# Autodesk Inventor assembly: POM_T5_01
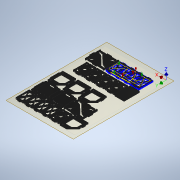
[picture p0: Inventor's stored thumbnail of the model, 180x180]
Saved by Autodesk Inventor 2020 (Build 240168000, 168)
## iProperties
Created: 2021-08-27
Part Number: POM_T5_01
Document SubType Name: Assembly
Designer: Masato
Author: Masato
## Documents named in this file (8)
- C:\Users\L20C1118 森　圭汰\Documents\220317_open\SUSTAINA-OP\Cam\POM_T5_01.iam
- C:\Users\L20C1118 森　圭汰\Documents\220317_open\SUSTAINA-OP\Cam\DisposableBoard.ipt
- C:\Users\L20C1118 森　圭汰\Documents\220317_open\SUSTAINA-OP\UpperBody\Head\Camera_root_frame.ipt
- C:\Users\L20C1118 森　圭汰\Documents\220317_open\SUSTAINA-OP\UpperBody\Head\Head_diagonal.ipt
- C:\Users\L20C1118 森　圭汰\Documents\220317_open\SUSTAINA-OP\UpperBody\Head\Head_horn_frame.ipt
- C:\Users\L20C1118 森　圭汰\Documents\220317_open\SUSTAINA-OP\UpperBody\Arm\ForeArm_diagonal.ipt
- C:\Users\L20C1118 森　圭汰\Documents\220317_open\SUSTAINA-OP\UpperBody\Head\Camera_side_frame.ipt
- C:\Users\L20C1118 森　圭汰\Documents\220317_open\SUSTAINA-OP\SandBlastingJig\Trunk_servo_bottom_frame_SandBlastingJig.ipt
## Components (29 placed, 7 different names)
1. DisposableBoard:1 — メイト:2, メイト:1, フラッシュ:1, フラッシュ:2, フラッシュ:3, フラッシュ:4, メイト:4, メイト:5, メイト:13, メイト:22, メイト:25, メイト:27, メイト:29, フラッシュ:12, フラッシュ:13, メイト:33, メイト:35, メイト:38, メイト:39, メイト:53, メイト:56, メイト:63, メイト:64, メイト:65, メイト:66, メイト:67
2. Camera_root_frame:1 — メイト:27, フラッシュ:11, メイト:41, メイト:48
3. Head_horn_frame:1 — メイト:29, フラッシュ:12, メイト:30, メイト:31, メイト:32
4. Camera_side_frame:1 — メイト:25, メイト:46, メイト:47, 正接:2
5. Camera_side_frame:2 — メイト:22, メイト:42, メイト:44, フラッシュ:14, メイト:47, メイト:52
6. ForeArm_diagonal:4 — フラッシュ:13, メイト:31, メイト:32, メイト:33, メイト:51
7. Camera_side_frame:3 — メイト:35, メイト:37, 正接:1, メイト:44, フラッシュ:14, メイト:51
8. Camera_side_frame:4 — メイト:37, 正接:1, メイト:38, メイト:46, 正接:2, メイト:55
9. Camera_root_frame:2 — メイト:39, メイト:41, メイト:42, メイト:49
10. Trunk_servo_bottom_frame_SandBlastingJig:1 — メイト:53, メイト:54, メイト:55, フラッシュ:15, メイト:57
11. Camera_side_frame:5 — メイト:66, フラッシュ:18
12. Camera_side_frame:6 — フラッシュ:17, メイト:65
13. Camera_side_frame:7 — メイト:62, メイト:63
14. Camera_side_frame:8 — メイト:64, メイト:68
15. Head_diagonal:2 — フラッシュ:3, フラッシュ:4, メイト:4, フラッシュ:5, メイト:6, フラッシュ:9, フラッシュ:11, メイト:48
16. Head_diagonal:1 — フラッシュ:5, メイト:5, メイト:6
17. Head_diagonal:3 — メイト:49
18. Head_diagonal:4 — メイト:30
19. ForeArm_diagonal:1 — メイト:13, フラッシュ:9, フラッシュ:17
20. ForeArm_diagonal:5
21. ForeArm_diagonal:6 — メイト:52, メイト:54
22. Head_horn_frame:2 — メイト:56, フラッシュ:15, メイト:57
23. Head_horn_frame:3
24. Head_horn_frame:4
25. Head_horn_frame:5 — メイト:62
26. Head_diagonal:5 — フラッシュ:18, メイト:67, メイト:68
27. Head_diagonal:6
28. Head_diagonal:7
29. Head_diagonal:8
## Component patterns: (2 elements, first: Head_diagonal:2 + Head_diagonal:1), (3 elements, first: ForeArm_diagonal:1), (4 elements, first: Head_horn_frame:2), (4 elements, first: Head_diagonal:5)
## Relationships (61: Mate 43, Flush 14, Tangent 4)
- メイト:2 [Mate]: DisposableBoard:1
- メイト:1 [Mate]: DisposableBoard:1
- フラッシュ:1 [Flush]: DisposableBoard:1
- フラッシュ:2 [Flush]: DisposableBoard:1
- フラッシュ:3 [Flush] (2 mm): DisposableBoard:1 ↔ Head_diagonal:2
- フラッシュ:4 [Flush] (2 mm): DisposableBoard:1 ↔ Head_diagonal:2
- メイト:4 [Mate]: DisposableBoard:1 ↔ Head_diagonal:2
- フラッシュ:5 [Flush]: Head_diagonal:2 ↔ Head_diagonal:1
- メイト:5 [Mate]: DisposableBoard:1 ↔ Head_diagonal:1
- メイト:6 [Mate] (2.5 mm): Head_diagonal:2 ↔ Head_diagonal:1
- メイト:13 [Mate]: DisposableBoard:1 ↔ ForeArm_diagonal:1
- フラッシュ:9 [Flush]: Head_diagonal:2 ↔ ForeArm_diagonal:1
- メイト:22 [Mate]: DisposableBoard:1 ↔ Camera_side_frame:2
- メイト:25 [Mate]: DisposableBoard:1 ↔ Camera_side_frame:1
- メイト:27 [Mate]: DisposableBoard:1 ↔ Camera_root_frame:1
- フラッシュ:11 [Flush]: Camera_root_frame:1 ↔ Head_diagonal:2
- メイト:29 [Mate]: DisposableBoard:1 ↔ Head_horn_frame:1
- フラッシュ:12 [Flush] (2 mm): DisposableBoard:1 ↔ Head_horn_frame:1
- フラッシュ:13 [Flush] (2 mm): DisposableBoard:1 ↔ ForeArm_diagonal:4
- メイト:30 [Mate] (2.5 mm): Head_horn_frame:1 ↔ Head_diagonal:4
- メイト:31 [Mate] (2.5 mm): Head_horn_frame:1 ↔ ForeArm_diagonal:4
- メイト:32 [Mate] (2.5 mm): Head_horn_frame:1 ↔ ForeArm_diagonal:4
- メイト:33 [Mate]: DisposableBoard:1 ↔ ForeArm_diagonal:4
- メイト:35 [Mate]: DisposableBoard:1 ↔ Camera_side_frame:3
- メイト:37 [Mate] (2.5 mm): Camera_side_frame:3 ↔ Camera_side_frame:4
- 正接:1 [Tangent] (2.5 mm): Camera_side_frame:3 ↔ Camera_side_frame:4
- メイト:38 [Mate]: DisposableBoard:1 ↔ Camera_side_frame:4
- メイト:39 [Mate]: DisposableBoard:1 ↔ Camera_root_frame:2
- メイト:41 [Mate] (2.5 mm): Camera_root_frame:1 ↔ Camera_root_frame:2
- メイト:42 [Mate] (2.5 mm): Camera_side_frame:2 ↔ Camera_root_frame:2
- メイト:44 [Mate] (2.5 mm): Camera_side_frame:2 ↔ Camera_side_frame:3
- フラッシュ:14 [Flush]: Camera_side_frame:2 ↔ Camera_side_frame:3
- メイト:46 [Mate] (2.5 mm): Camera_side_frame:1 ↔ Camera_side_frame:4
- メイト:47 [Mate] (2.5 mm): Camera_side_frame:1 ↔ Camera_side_frame:2
- 正接:2 [Tangent] (2.5 mm): Camera_side_frame:1 ↔ Camera_side_frame:4
- メイト:48 [Mate] (2.5 mm): Camera_root_frame:1 ↔ Head_diagonal:2
- メイト:49 [Mate] (2.5 mm): Camera_root_frame:2 ↔ Head_diagonal:3
- メイト:51 [Mate] (2.5 mm): ForeArm_diagonal:4 ↔ Camera_side_frame:3
- メイト:52 [Mate] (2.5 mm): Camera_side_frame:2 ↔ ForeArm_diagonal:6
- メイト:53 [Mate]: DisposableBoard:1 ↔ Trunk_servo_bottom_frame_SandBlastingJig:1
- メイト:54 [Mate] (6 mm): Trunk_servo_bottom_frame_SandBlastingJig:1 ↔ ForeArm_diagonal:6
- メイト:55 [Mate] (70 mm): Camera_side_frame:4 ↔ Trunk_servo_bottom_frame_SandBlastingJig:1
- メイト:56 [Mate]: DisposableBoard:1 ↔ Head_horn_frame:2
- フラッシュ:15 [Flush]: Trunk_servo_bottom_frame_SandBlastingJig:1 ↔ Head_horn_frame:2
- メイト:57 [Mate] (2.5 mm): Trunk_servo_bottom_frame_SandBlastingJig:1 ↔ Head_horn_frame:2
- [Mate] (2.5 mm): Camera_side_frame:7 ↔ Camera_side_frame:8
- [Tangent] (2.5 mm): Camera_side_frame:7 ↔ Camera_side_frame:8
- [Mate] (2.5 mm): Camera_side_frame:6 ↔ Camera_side_frame:7
- [Flush]: Camera_side_frame:6 ↔ Camera_side_frame:7
- [Mate] (2.5 mm): Camera_side_frame:5 ↔ Camera_side_frame:8
- [Mate] (2.5 mm): Camera_side_frame:5 ↔ Camera_side_frame:6
- [Tangent] (2.5 mm): Camera_side_frame:5 ↔ Camera_side_frame:8
- フラッシュ:17 [Flush]: Camera_side_frame:6 ↔ ForeArm_diagonal:1
- メイト:62 [Mate] (5 mm): Camera_side_frame:7 ↔ Head_horn_frame:5
- メイト:63 [Mate]: DisposableBoard:1 ↔ Camera_side_frame:7
- メイト:64 [Mate]: DisposableBoard:1 ↔ Camera_side_frame:8
- メイト:65 [Mate]: DisposableBoard:1 ↔ Camera_side_frame:6
- メイト:66 [Mate]: DisposableBoard:1 ↔ Camera_side_frame:5
- フラッシュ:18 [Flush]: Camera_side_frame:5 ↔ Head_diagonal:5
- メイト:67 [Mate]: DisposableBoard:1 ↔ Head_diagonal:5
- メイト:68 [Mate] (2.5 mm): Camera_side_frame:8 ↔ Head_diagonal:5
## Named parameters: d159_d132 = 2.5 mm, d160_d134 = 0 mm, d161_d135 = 2.5 mm, d162_d136 = 2.5 mm, d163_d137 = 2.5 mm, d164_d122 = 2.5 mm, d165_d123 = 2.5 mm
